# Autodesk Inventor assembly: Entrada
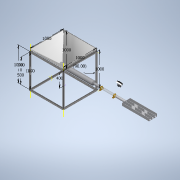
[picture p0: Inventor's stored thumbnail of the model, 180x180]
Saved by Autodesk Inventor 2020 (Build 240168000, 168)
## iProperties
_SolveAssemblyDoc: Frame Generator Solve Assembly
_Version: 15.0.0
Created: 2020-02-17
Part Number: Entrada
Material: Genérico
Document SubType Name: Assembly
Designer: PabloGod
Author: PabloGod
## Documents named in this file (12)
- D:\Tesis\Entrada.iam
- D:\Tesis\Tubo tolba.ipt
- D:\Tesis\Tolba para Sembradora manual.ipt
- D:\Tesis\armadura de tolba.ipt
- D:\Tesis\Tubor reduccion.ipt
- D:\Tesis\tubo transparente.ipt
- D:\Tesis\Tubo pre distribucion.ipt
- D:\Tesis\Abrazaderas tubo transparente.ipt
- D:\Tesis\Camara.ipt
- D:\Tesis\Barra LED Machine Vision.ipt
- D:\Tesis\Distribuidor de truchas.ipt
- D:\Tesis\Entrada\Frame\Frame 1582651521180.iam
## Components (12 placed, 11 different names)
1. Tubo tolba:1 — Nivelación:1, Coincidencia:9, Coincidencia:10
2. Armadura de tolba:1
3. Tolba para Sembradora manual:1 — Coincidencia:1, Coincidencia:2
4. Tubor reduccion:1 — Coincidencia:9, Coincidencia:10, Coincidencia:11, Coincidencia:12
5. Contadora y clasificadora:1 — Coincidencia:11, Coincidencia:12, Coincidencia:13, Coincidencia:14, Coincidencia:15, Coincidencia:17, Coincidencia:18, Nivelación:4
6. Tubo pre distribucion:1 — Coincidencia:13, Coincidencia:14, Insertar:1
7. Abrazaderas tubo transparente:1 — Coincidencia:18, Nivelación:4
8. Abrazaderas tubo transparente:2 — Coincidencia:15, Coincidencia:17
9. Camara:1 — Coincidencia:19, Nivelación:5
10. Barra LED Machine Vision:1 — Coincidencia:19, Nivelación:5
11. Distribuidor de truchas:1 — Insertar:1
12. Frame 1582651521180:1 [sub-assembly]
## Relationships (20: Mate 14, Flush 5, Insert 1)
- Nivelación:1 [Flush]: Tubo tolba:1
- Nivelación:2 [Flush] (40 mm)
- Coincidencia:1 [Mate]: Tolba para Sembradora manual:1
- Coincidencia:2 [Mate]: Tolba para Sembradora manual:1
- Nivelación:3 [Flush] (350 mm)
- Coincidencia:6 [Mate]
- Coincidencia:8 [Mate]
- Coincidencia:9 [Mate]: Tubo tolba:1 ↔ Tubor reduccion:1
- Coincidencia:10 [Mate]: Tubo tolba:1 ↔ Tubor reduccion:1
- Coincidencia:11 [Mate]: Tubor reduccion:1 ↔ Contadora y clasificadora:1
- Coincidencia:12 [Mate]: Tubor reduccion:1 ↔ Contadora y clasificadora:1
- Coincidencia:13 [Mate]: Contadora y clasificadora:1 ↔ Tubo pre distribucion:1
- Coincidencia:14 [Mate]: Contadora y clasificadora:1 ↔ Tubo pre distribucion:1
- Coincidencia:15 [Mate]: Contadora y clasificadora:1 ↔ Abrazaderas tubo transparente:2
- Coincidencia:17 [Mate] (-15 mm): Contadora y clasificadora:1 ↔ Abrazaderas tubo transparente:2
- Coincidencia:18 [Mate]: Contadora y clasificadora:1 ↔ Abrazaderas tubo transparente:1
- Nivelación:4 [Flush] (-15 mm): Contadora y clasificadora:1 ↔ Abrazaderas tubo transparente:1
- Coincidencia:19 [Mate]: Camara:1 ↔ Barra LED Machine Vision:1
- Nivelación:5 [Flush]: Camara:1 ↔ Barra LED Machine Vision:1
- Insertar:1: Tubo pre distribucion:1 ↔ Distribuidor de truchas:1
